# Autodesk Inventor assembly: lazysusan2
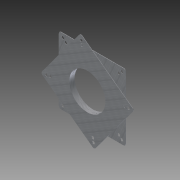
[picture p0: Inventor's stored thumbnail of the model, 180x180]
Saved by Autodesk Inventor 2011 (Build 150239000, 239)
## iProperties
Created: 2011-09-17
Part Number: lazysusan2
Document SubType Name: Assembly
Designer: Matthew
Author: Matthew
## Documents named in this file (2)
- C:\Users\Matthew\Documents\matthew_autocad\prlite\lazy susan\lazysusan2.iam
- C:\Users\Matthew\Documents\matthew_autocad\prlite\lazy susan\3.ipt
## Components (2 placed, 1 different names)
1. 3:1 — Mate:1, Mate:2
2. 3:2 — Mate:1, Mate:2
## Relationships (2: Mate 2)
- Mate:1: 3:1 ↔ 3:2
- Mate:2: 3:1 ↔ 3:2
